# Autodesk Inventor assembly: Intake
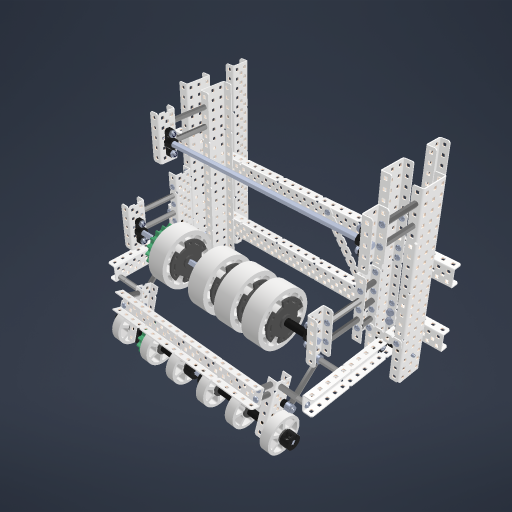
[picture p0: Inventor's stored thumbnail of the model, 512x512]
Saved by Autodesk Inventor 2023 (Build 270158000, 158)
## iProperties
Created: 2022-09-02
Part Number: Intake
Document SubType Name: Assembly
Designer: alex
Author: alex
## Documents named in this file (43)
- C:\Users\alex\Documents\GitHub\4067X_spin_up_cad\Mechanism\Intake.iam
- C:\Users\alex\Documents\GitHub\4067X_spin_up_cad\Library\Structure\Standoff\Standoff 1.00.ipt
- C:\Users\alex\Documents\GitHub\4067X_spin_up_cad\Library\Structure\Standoff.ipt
- C:\Users\alex\Documents\GitHub\4067X_spin_up_cad\Library\Structure\Hardware\Screw Steel - Star\SScrew Star Smooth .290.ipt
- C:\Users\alex\Documents\GitHub\4067X_spin_up_cad\Library\Structure\Hardware\Screw Steel - Star.ipt
- C:\Users\alex\Documents\GitHub\4067X_spin_up_cad\Library\Structure\Standoff\Standoff .50.ipt
- C:\Users\alex\Documents\GitHub\4067X_spin_up_cad\Library\Motion\Spacers\Spacer Nylon .375 OD.ipt
- C:\Users\alex\Documents\GitHub\4067X_spin_up_cad\Library\Structure\Hardware\Nut Keps.ipt
- C:\Users\alex\Documents\GitHub\4067X_spin_up_cad\Library\Structure\Hardware\Screw Steel - Star\SScrew Star Smooth .375.ipt
- C:\Users\alex\Documents\GitHub\4067X_spin_up_cad\Library\Structure\C-Channels\Aluminum 1x3x1\Alu C 1x3x1x20.ipt
- C:\Users\alex\Documents\GitHub\4067X_spin_up_cad\Library\Structure\C-Channels\Aluminum 1x3x1\Alu C 1x3x1x5.ipt
- C:\Users\alex\Documents\GitHub\4067X_spin_up_cad\Library\Structure\C-Channels\Aluminum 1x2x1\Alu C 1x2x1x35.ipt
- C:\Users\alex\Documents\GitHub\4067X_spin_up_cad\Library\Structure\Plates\Aluminum\VEX Plates\Alu Plate VEX 1x11.ipt
- C:\Users\alex\Documents\GitHub\4067X_spin_up_cad\Library\Structure\Standoff\Standoff 2.00.ipt
- C:\Users\alex\Documents\GitHub\4067X_spin_up_cad\Library\Structure\C-Channels\Aluminum 1x2x1\Alu C 1x2x1x5.ipt
- C:\Users\alex\Documents\GitHub\4067X_spin_up_cad\Library\Structure\C-Channels\Aluminum 1x2x1\Alu C 1x2x1x7.ipt
- C:\Users\alex\Documents\GitHub\4067X_spin_up_cad\Library\Structure\Standoff\Standoff .75.ipt
- C:\Users\alex\Documents\GitHub\4067X_spin_up_cad\Library\Motion\Spacers\Spacer Nylon .375 OD\NSpacer .375 OD x .125.ipt
- C:\Users\alex\Documents\GitHub\4067X_spin_up_cad\Library\Motion\Shaft HS\HS Bearing Flat.ipt
- C:\Users\alex\Documents\GitHub\4067X_spin_up_cad\Library\Structure\Hardware\Nut Thin Nylock.ipt
- C:\Users\alex\Documents\GitHub\4067X_spin_up_cad\Library\Structure\Hardware\Screw Steel - Star\SScrew Star Smooth .500.ipt
- C:\Users\alex\Documents\GitHub\4067X_spin_up_cad\Library\Motion\Shaft HS\Shaft HS\Shaft HS 12.0 in.ipt
- C:\Users\alex\Documents\GitHub\4067X_spin_up_cad\Library\Motion\Shaft HS\Shaft HS.ipt
- C:\Users\alex\Documents\GitHub\4067X_spin_up_cad\Library\Motion\Shaft HS\HS Spacer.ipt
- C:\Users\alex\Documents\GitHub\4067X_spin_up_cad\3FlexWheel.iam
- C:\Users\alex\Documents\GitHub\4067X_spin_up_cad\Library\Motion\Shaft HS\HS Spacer\HSpacer .2500.ipt
- C:\Users\alex\Documents\GitHub\4067X_spin_up_cad\Library\Motion\Sprockets\HS 18T Sprocket, No Insert.ipt
- C:\Users\alex\Documents\GitHub\4067X_spin_up_cad\Library\Structure\Hardware\Screw Steel - Star\SScrew Star Smooth 2.250.ipt
- C:\Users\alex\Documents\GitHub\4067X_spin_up_cad\Mechanism\FloatingIntake.iam
- C:\Users\alex\Documents\GitHub\4067X_spin_up_cad\Library\Motion\Spacers\Spacer Nylon .375 OD\NSpacer .375 OD x .375.ipt
- C:\Users\alex\Documents\GitHub\4067X_spin_up_cad\Library\Motion\Spacers\Washer Steel\SWasher .375 OD x .015625.ipt
- C:\Users\alex\Documents\GitHub\4067X_spin_up_cad\Library\Motion\Spacers\Washer Steel.ipt
- C:\Users\alex\Documents\GitHub\4067X_spin_up_cad\Library\Motion\1-Post Bearing Flat Hex Retainer.ipt
- C:\Users\alex\Documents\GitHub\4067X_spin_up_cad\Library\Structure\Hardware\Nut Nylock.ipt
- C:\Users\alex\Documents\GitHub\4067X_spin_up_cad\Library\Motion\Spacers\Spacer Nylon .375 OD\NSpacer .375 OD x .500.ipt
- C:\Users\alex\Documents\GitHub\4067X_spin_up_cad\Library\Motion\Spacers\Washer Teflon\TWasher .375 OD x .06250.ipt
- C:\Users\alex\Documents\GitHub\4067X_spin_up_cad\Library\Motion\Spacers\Washer Teflon.ipt
- C:\Users\alex\Documents\GitHub\4067X_spin_up_cad\Library\Motion\Shaft HS\HS Shaft Collar.ipt
- C:\Users\alex\Documents\GitHub\4067X_spin_up_cad\Library\Motion\Shaft HS\HS Spacer\HSpacer .5000.ipt
- C:\Users\alex\Documents\GitHub\4067X_spin_up_cad\Library\Motion\Shaft HS\HS Spacer\HSpacer .1250.ipt
- C:\Users\alex\Documents\GitHub\4067X_spin_up_cad\Library\Structure\C-Channels\Aluminum 1x2x1\Alu C 1x2x1x21.ipt
- C:\Users\alex\Documents\GitHub\4067X_spin_up_cad\Library\Structure\Hardware\Screw Steel - Star\SScrew Star Smooth .750.ipt
- C:\Users\alex\Documents\GitHub\4067X_spin_up_cad\Library\Structure\Plates\Aluminum\VEX Plates\Alu Plate VEX 1x4.ipt
## Components (166 placed, 35 different names)
1. Alu C 1x2x1x35:1 — Insert:150, Insert:151, Insert:218, Insert:219, Insert:236, Insert:237, Insert:400, Insert:401, Insert:419, Insert:420, Insert:448, Insert:449, Insert:458, Insert:459, Insert:469, Insert:475, Insert:504, Insert:505
2. Standoff 1.00:16 — Insert:110, Insert:404
3. Standoff .50:17 — Insert:110, Insert:496
4. Standoff 1.00:18 — Insert:405
5. Standoff .50:19 — Insert:497
6. Standoff 1.00:20 — Insert:454
7. Standoff .50:21 — Insert:500
8. Standoff 1.00:22 — Insert:455
9. Standoff .50:23 — Insert:501
10. Alu C 1x3x1x5:2 — Insert:150, Insert:151, Insert:217, Insert:220, Insert:221, Insert:428, Mate:67, Insert:429, Insert:439
11. Nut Keps:12 — Insert:217
12. SScrew Star Smooth .290:52 — Insert:218
13. SScrew Star Smooth .290:53 — Insert:219
14. Nut Keps:13 — Insert:220
15. Nut Keps:14 — Insert:221
16. SScrew Star Smooth .290:62 — Insert:236
17. SScrew Star Smooth .290:63 — Insert:237
18. Alu C 1x2x1x35:2 — Insert:417, Insert:418, Insert:467, Insert:470, Insert:476, Insert:481, Insert:482, Insert:535, Insert:536
19. SScrew Star Smooth .290:86 — Insert:456
20. SScrew Star Smooth .290:90 — Insert:407
21. SScrew Star Smooth .290:91 — Insert:406
22. Alu C 1x2x1x5:2 — Insert:334, Insert:335, Insert:338, Insert:339, Insert:488, Mate:72, Insert:489, Insert:490
23. Standoff 2.00:27 — Insert:334, Insert:382
24. Standoff 2.00:28 — Insert:335, Insert:381
25. SScrew Star Smooth .290:102 — Insert:338
26. SScrew Star Smooth .290:103 — Insert:339
27. Alu C 1x2x1x7:1 — Insert:345, Insert:346, Insert:347, Insert:348, Insert:349, Insert:358, Insert:359, Insert:360, Insert:361, Insert:362, Insert:381, Insert:382, Insert:522
28. SScrew Star Smooth .290:106 — Insert:345
29. SScrew Star Smooth .290:107 — Insert:346
30. Standoff .75:29 — Insert:347, Insert:355
31. Standoff .75:30 — Insert:348, Insert:356
32. Standoff .75:31 — Insert:349, Insert:357
33. NSpacer .375 OD x .125:13 — Insert:355
34. NSpacer .375 OD x .125:14 — Insert:356
35. NSpacer .375 OD x .125:15 — Insert:357
36. SScrew Star Smooth .375:111 — Insert:358
37. SScrew Star Smooth .375:112 — Insert:359
38. SScrew Star Smooth .375:113 — Insert:360
39. SScrew Star Smooth .290:114 — Insert:361
40. SScrew Star Smooth .290:115 — Insert:362
41. Alu C 1x2x1x5:3 — Insert:485, Mate:71, Insert:486, Insert:487, Flush:1
42. Standoff 2.00:32 — Insert:384
43. Standoff 2.00:33 — Insert:383
44. SScrew Star Smooth .290:116
45. SScrew Star Smooth .290:117
46. Alu C 1x2x1x7:2 — Insert:383, Insert:384, Insert:521, Mate:77, Insert:528, Insert:529
47. SScrew Star Smooth .290:118
48. Standoff .75:34
49. Standoff .75:35
50. Standoff .75:36
51. NSpacer .375 OD x .125:16
52. NSpacer .375 OD x .125:17
53. NSpacer .375 OD x .125:18
54. SScrew Star Smooth .375:120
55. SScrew Star Smooth .375:121
56. SScrew Star Smooth .375:122
57. SScrew Star Smooth .290:123
58. SScrew Star Smooth .290:124
59. Shaft HS 12.0 in:1 — Mate:43, Angle:1, Angle:2, Mate:47, Mate:50, Mate:51, Mate:53, Angle:3, Mate:57, Angle:4, Mate:58, Angle:5, Mate:73, Flush:1, Mate:74
60. 3FlexWheel:1 [sub-assembly] — Mate:43, Angle:1, Mate:48, Mate:76
61. 3FlexWheel:2 [sub-assembly] — Angle:2, Mate:49, Mate:50, Mate:52
62. HSpacer .2500:2 — Mate:47, Mate:48, Mate:49
63. HSpacer .2500:3 — Mate:51, Mate:52, Mate:54
64. 3FlexWheel:3 [sub-assembly] — Mate:53, Angle:3, Mate:54
65. 3FlexWheel:4 [sub-assembly] — Mate:58, Angle:5, Mate:59
66. HS 18T Sprocket, No Insert:1 — Mate:57, Angle:4, Mate:59, Flush:2, Mate:75
67. Alu C 1x3x1x20:3 — Insert:400, Insert:401, Insert:404, Insert:405, Insert:406, Insert:407, Insert:413, Insert:414, Insert:416, Insert:460, Insert:461, Insert:467, Insert:468, Insert:521, Insert:527, Insert:530, Insert:531, Insert:532
68. SScrew Star Smooth 2.250:132 — Insert:413
69. Nut Keps:43 — Insert:414, Insert:433
70. SScrew Star Smooth .290:134 — Insert:416
71. Nut Keps:44 — Insert:417
72. Nut Keps:45 — Insert:418
73. Alu C 1x3x1x20:4 — Insert:419, Insert:420, Insert:421, Insert:424, Mate:66, Insert:446, Insert:452, Insert:453, Insert:454, Insert:455, Insert:456, Insert:457, Insert:462, Insert:463, Insert:479, Insert:480, Insert:522, Insert:523
74. SScrew Star Smooth 2.250:135 — Insert:421, Mate:65
75. Nut Keps:46 — Insert:424, Insert:425
76. FloatingIntake:1 [sub-assembly] — Mate:65, Mate:66, Insert:430, Insert:435, Flush:2
77. NSpacer .375 OD x .375:19 — Insert:425, Insert:426
78. SWasher .375 OD x .015625:1 — Insert:426
79. 1-Post Bearing Flat Hex Retainer:1 — Insert:428, Mate:67
80. Nut Nylock:1
81. SScrew Star Smooth .375:136 — Insert:429
82. NSpacer .375 OD x .500:20 — Insert:430, Insert:431
83. NSpacer .375 OD x .375:21 — Insert:431
84. NSpacer .375 OD x .375:22 — Insert:433
85. SWasher .375 OD x .015625:2
86. NSpacer .375 OD x .500:23 — Insert:435
87. NSpacer .375 OD x .375:24
88. TWasher .375 OD x .06250:1 — Insert:439
89. SScrew Star Smooth .375:138
90. TWasher .375 OD x .06250:2 — Insert:524, Insert:525
91. SScrew Star Smooth .375:139
92. Nut Keps:47 — Insert:446
93. SScrew Star Smooth .290:141 — Insert:448
94. SScrew Star Smooth .290:142 — Insert:449
95. Nut Keps:50 — Insert:452
96. Nut Keps:51 — Insert:453
97. SScrew Star Smooth .290:143 — Insert:457
98. SScrew Star Smooth .290:144 — Insert:458
99. SScrew Star Smooth .290:145 — Insert:459
100. Nut Keps:52 — Insert:460
101. Nut Keps:53 — Insert:461
102. SScrew Star Smooth .290:146 — Insert:462
103. SScrew Star Smooth .290:147 — Insert:463
104. SScrew Star Smooth .290:149 — Insert:468
105. Alu Plate VEX 1x11:4 — Insert:469, Insert:470, Insert:473, Insert:474
106. SScrew Star Smooth .290:152 — Insert:473
107. SScrew Star Smooth .290:153 — Insert:474
108. Nut Keps:54 — Insert:475
109. Nut Keps:55 — Insert:476
110. SScrew Star Smooth .290:154 — Insert:479
111. SScrew Star Smooth .290:155 — Insert:480
112. Nut Keps:58 — Insert:481
113. Nut Keps:59 — Insert:482
114. HS Bearing Flat:3 — Insert:485, Mate:71, Insert:493
115. Nut Thin Nylock:5
116. Nut Thin Nylock:6
117. SScrew Star Smooth .500:156 — Insert:486
118. SScrew Star Smooth .500:157 — Insert:487
119. HS Bearing Flat:4 — Insert:488, Mate:72, Mate:73, Insert:491, Insert:492
120. SScrew Star Smooth .500:158 — Insert:489
121. SScrew Star Smooth .500:159 — Insert:490
122. Nut Thin Nylock:7 — Insert:491
123. Nut Thin Nylock:8 — Insert:492
124. HS Shaft Collar:1 — Mate:74, Mate:75
125. HSpacer .5000:4 — Insert:493, Insert:494
126. HSpacer .5000:5 — Insert:494, Insert:495
127. HSpacer .1250:6 — Insert:495, Mate:76
128. Alu C 1x2x1x21:1 — Insert:496, Insert:497, Insert:498, Insert:499
129. SScrew Star Smooth .750:160 — Insert:498
130. SScrew Star Smooth .750:161 — Insert:499
131. Alu C 1x2x1x21:2 — Insert:500, Insert:501, Insert:502, Insert:503
132. SScrew Star Smooth .750:162 — Insert:502
133. SScrew Star Smooth .750:163 — Insert:503
134. Alu C 1x3x1x20:5 — Insert:504, Insert:505, Insert:506, Insert:507, Insert:508, Insert:525, Insert:541, Insert:542
135. Nut Keps:60 — Insert:506
136. Nut Keps:61 — Insert:507
137. Nut Keps:62 — Insert:508
138. Alu C 1x2x1x5:5 — Insert:545, Mate:78, Insert:546, Insert:547
139. Standoff 2.00:39 — Insert:541
140. Standoff 2.00:40 — Insert:542
141. SScrew Star Smooth .290:166
142. SScrew Star Smooth .290:167
143. SScrew Star Smooth .290:168 — Insert:523
144. Alu Plate VEX 1x4:1 — Insert:524, Mate:77, Insert:526
145. SScrew Star Smooth .375:169 — Insert:526
146. Nut Keps:64 — Insert:527
147. SScrew Star Smooth .290:170 — Insert:528
148. SScrew Star Smooth .290:171 — Insert:529
149. Nut Keps:65 — Insert:530
150. Nut Keps:66 — Insert:531
151. Nut Keps:67 — Insert:532
152. Alu C 1x3x1x20:6 — Insert:535, Insert:536, Insert:539, Insert:540
153. Alu C 1x2x1x5:6 — Insert:550, Mate:79, Insert:551, Insert:552, Flush:3
154. Standoff 2.00:41 — Insert:539
155. Standoff 2.00:42 — Insert:540
156. HS Bearing Flat:5 — Insert:545, Mate:78
157. Nut Thin Nylock:9
158. Nut Thin Nylock:10
159. SScrew Star Smooth .500:172 — Insert:546
160. SScrew Star Smooth .500:173 — Insert:547
161. HS Bearing Flat:6 — Insert:550, Mate:79, Mate:80
162. Nut Thin Nylock:11
163. Nut Thin Nylock:12
164. SScrew Star Smooth .500:174 — Insert:551
165. SScrew Star Smooth .500:175 — Insert:552
166. Shaft HS 12.0 in:2 — Mate:80, Flush:3
## Relationships (197: Insert 164, Mate 25, Angle 5, Flush 3)
- Insert:110: Standoff 1.00:16 ↔ Standoff .50:17
- [Insert]: Standoff 1.00:18 ↔ Standoff .50:19
- [Insert]: Standoff 1.00:20 ↔ Standoff .50:21
- [Insert]: Standoff 1.00:22 ↔ Standoff .50:23
- Insert:150: Alu C 1x2x1x35:1 ↔ Alu C 1x3x1x5:2
- Insert:151: Alu C 1x2x1x35:1 ↔ Alu C 1x3x1x5:2
- Insert:217: Alu C 1x3x1x5:2 ↔ Nut Keps:12
- Insert:218: Alu C 1x2x1x35:1 ↔ SScrew Star Smooth .290:52
- Insert:219: Alu C 1x2x1x35:1 ↔ SScrew Star Smooth .290:53
- Insert:220: Alu C 1x3x1x5:2 ↔ Nut Keps:13
- Insert:221: Alu C 1x3x1x5:2 ↔ Nut Keps:14
- Insert:236: Alu C 1x2x1x35:1 ↔ SScrew Star Smooth .290:62
- Insert:237: Alu C 1x2x1x35:1 ↔ SScrew Star Smooth .290:63
- Insert:334: Alu C 1x2x1x5:2 ↔ Standoff 2.00:27
- Insert:335: Alu C 1x2x1x5:2 ↔ Standoff 2.00:28
- Insert:338: Alu C 1x2x1x5:2 ↔ SScrew Star Smooth .290:102
- Insert:339: Alu C 1x2x1x5:2 ↔ SScrew Star Smooth .290:103
- Insert:345: Alu C 1x2x1x7:1 ↔ SScrew Star Smooth .290:106
- Insert:346: Alu C 1x2x1x7:1 ↔ SScrew Star Smooth .290:107
- Insert:347: Alu C 1x2x1x7:1 ↔ Standoff .75:29
- Insert:348: Alu C 1x2x1x7:1 ↔ Standoff .75:30
- Insert:349: Alu C 1x2x1x7:1 ↔ Standoff .75:31
- Insert:355: Standoff .75:29 ↔ NSpacer .375 OD x .125:13
- Insert:356: Standoff .75:30 ↔ NSpacer .375 OD x .125:14
- Insert:357: Standoff .75:31 ↔ NSpacer .375 OD x .125:15
- Insert:358: Alu C 1x2x1x7:1 ↔ SScrew Star Smooth .375:111
- Insert:359: Alu C 1x2x1x7:1 ↔ SScrew Star Smooth .375:112
- Insert:360: Alu C 1x2x1x7:1 ↔ SScrew Star Smooth .375:113
- Insert:361: Alu C 1x2x1x7:1 ↔ SScrew Star Smooth .290:114
- Insert:362: Alu C 1x2x1x7:1 ↔ SScrew Star Smooth .290:115
- [Insert]: Alu C 1x2x1x5:3 ↔ Standoff 2.00:32
- [Insert]: Alu C 1x2x1x5:3 ↔ Standoff 2.00:33
- [Insert]: Alu C 1x2x1x5:3 ↔ SScrew Star Smooth .290:116
- [Insert]: Alu C 1x2x1x5:3 ↔ SScrew Star Smooth .290:117
- [Insert]: Alu C 1x2x1x7:2 ↔ SScrew Star Smooth .290:118
- [Insert]: Alu C 1x2x1x7:2 ↔ Standoff .75:34
- [Insert]: Alu C 1x2x1x7:2 ↔ Standoff .75:35
- [Insert]: Alu C 1x2x1x7:2 ↔ Standoff .75:36
- [Insert]: Standoff .75:34 ↔ NSpacer .375 OD x .125:16
- [Insert]: Standoff .75:35 ↔ NSpacer .375 OD x .125:17
- [Insert]: Standoff .75:36 ↔ NSpacer .375 OD x .125:18
- [Insert]: Alu C 1x2x1x7:2 ↔ SScrew Star Smooth .375:120
- [Insert]: Alu C 1x2x1x7:2 ↔ SScrew Star Smooth .375:121
- [Insert]: Alu C 1x2x1x7:2 ↔ SScrew Star Smooth .375:122
- [Insert]: Alu C 1x2x1x7:2 ↔ SScrew Star Smooth .290:123
- [Insert]: Alu C 1x2x1x7:2 ↔ SScrew Star Smooth .290:124
- Insert:381: Standoff 2.00:28 ↔ Alu C 1x2x1x7:1
- Insert:382: Standoff 2.00:27 ↔ Alu C 1x2x1x7:1
- Insert:383: Standoff 2.00:33 ↔ Alu C 1x2x1x7:2
- Insert:384: Standoff 2.00:32 ↔ Alu C 1x2x1x7:2
- Mate:43: Shaft HS 12.0 in:1 ↔ 3FlexWheel:1
- Angle:1 (0 deg): Shaft HS 12.0 in:1 ↔ 3FlexWheel:1
- Angle:2 (0 deg): Shaft HS 12.0 in:1 ↔ 3FlexWheel:2
- Mate:47: Shaft HS 12.0 in:1 ↔ HSpacer .2500:2
- Mate:48: 3FlexWheel:1 ↔ HSpacer .2500:2
- Mate:49: 3FlexWheel:2 ↔ HSpacer .2500:2
- Mate:50: Shaft HS 12.0 in:1 ↔ 3FlexWheel:2
- Mate:51: Shaft HS 12.0 in:1 ↔ HSpacer .2500:3
- Mate:52: 3FlexWheel:2 ↔ HSpacer .2500:3
- Mate:53: Shaft HS 12.0 in:1 ↔ 3FlexWheel:3
- Angle:3 (0 deg): Shaft HS 12.0 in:1 ↔ 3FlexWheel:3
- Mate:54: HSpacer .2500:3 ↔ 3FlexWheel:3
- Mate:57: Shaft HS 12.0 in:1 ↔ HS 18T Sprocket, No Insert:1
- Angle:4 (0 deg): Shaft HS 12.0 in:1 ↔ HS 18T Sprocket, No Insert:1
- Mate:58: Shaft HS 12.0 in:1 ↔ 3FlexWheel:4
- Angle:5 (0 deg): Shaft HS 12.0 in:1 ↔ 3FlexWheel:4
- Mate:59: 3FlexWheel:4 ↔ HS 18T Sprocket, No Insert:1
- Insert:400: Alu C 1x2x1x35:1 ↔ Alu C 1x3x1x20:3
- Insert:401: Alu C 1x2x1x35:1 ↔ Alu C 1x3x1x20:3
- Insert:404: Standoff 1.00:16 ↔ Alu C 1x3x1x20:3
- Insert:405: Standoff 1.00:18 ↔ Alu C 1x3x1x20:3
- Insert:406: SScrew Star Smooth .290:91 ↔ Alu C 1x3x1x20:3
- Insert:407: SScrew Star Smooth .290:90 ↔ Alu C 1x3x1x20:3
- Insert:413: Alu C 1x3x1x20:3 ↔ SScrew Star Smooth 2.250:132
- Insert:414: Alu C 1x3x1x20:3 ↔ Nut Keps:43
- Insert:416: Alu C 1x3x1x20:3 ↔ SScrew Star Smooth .290:134
- Insert:417: Alu C 1x2x1x35:2 ↔ Nut Keps:44
- Insert:418: Alu C 1x2x1x35:2 ↔ Nut Keps:45
- Insert:419: Alu C 1x2x1x35:1 ↔ Alu C 1x3x1x20:4
- Insert:420: Alu C 1x2x1x35:1 ↔ Alu C 1x3x1x20:4
- Insert:421: Alu C 1x3x1x20:4 ↔ SScrew Star Smooth 2.250:135
- Insert:424: Alu C 1x3x1x20:4 ↔ Nut Keps:46
- Mate:65: SScrew Star Smooth 2.250:135 ↔ FloatingIntake:1
- Mate:66 (13.6398 mm): Alu C 1x3x1x20:4 ↔ FloatingIntake:1
- Insert:425: Nut Keps:46 ↔ NSpacer .375 OD x .375:19
- Insert:426: NSpacer .375 OD x .375:19 ↔ SWasher .375 OD x .015625:1
- [Insert]: 1-Post Bearing Flat Hex Retainer:1 ↔ Nut Nylock:1
- Insert:428: Alu C 1x3x1x5:2 ↔ 1-Post Bearing Flat Hex Retainer:1
- Mate:67: Alu C 1x3x1x5:2 ↔ 1-Post Bearing Flat Hex Retainer:1
- Insert:429: Alu C 1x3x1x5:2 ↔ SScrew Star Smooth .375:136
- Insert:430: FloatingIntake:1 ↔ NSpacer .375 OD x .500:20
- Insert:431: NSpacer .375 OD x .500:20 ↔ NSpacer .375 OD x .375:21
- [Insert]: NSpacer .375 OD x .375:22 ↔ SWasher .375 OD x .015625:2
- Insert:433: Nut Keps:43 ↔ NSpacer .375 OD x .375:22
- [Insert]: NSpacer .375 OD x .500:23 ↔ NSpacer .375 OD x .375:24
- Insert:435: FloatingIntake:1 ↔ NSpacer .375 OD x .500:23
- Insert:439: Alu C 1x3x1x5:2 ↔ TWasher .375 OD x .06250:1
- Insert:446: Alu C 1x3x1x20:4 ↔ Nut Keps:47
- Insert:448: Alu C 1x2x1x35:1 ↔ SScrew Star Smooth .290:141
- Insert:449: Alu C 1x2x1x35:1 ↔ SScrew Star Smooth .290:142
- Insert:452: Alu C 1x3x1x20:4 ↔ Nut Keps:50
- Insert:453: Alu C 1x3x1x20:4 ↔ Nut Keps:51
- Insert:454: Standoff 1.00:20 ↔ Alu C 1x3x1x20:4
- Insert:455: Standoff 1.00:22 ↔ Alu C 1x3x1x20:4
- Insert:456: SScrew Star Smooth .290:86 ↔ Alu C 1x3x1x20:4
- Insert:457: Alu C 1x3x1x20:4 ↔ SScrew Star Smooth .290:143
- Insert:458: Alu C 1x2x1x35:1 ↔ SScrew Star Smooth .290:144
- Insert:459: Alu C 1x2x1x35:1 ↔ SScrew Star Smooth .290:145
- Insert:460: Alu C 1x3x1x20:3 ↔ Nut Keps:52
- Insert:461: Alu C 1x3x1x20:3 ↔ Nut Keps:53
- Insert:462: Alu C 1x3x1x20:4 ↔ SScrew Star Smooth .290:146
- Insert:463: Alu C 1x3x1x20:4 ↔ SScrew Star Smooth .290:147
- Insert:467: Alu C 1x2x1x35:2 ↔ Alu C 1x3x1x20:3
- Insert:468: Alu C 1x3x1x20:3 ↔ SScrew Star Smooth .290:149
- Insert:469: Alu C 1x2x1x35:1 ↔ Alu Plate VEX 1x11:4
- Insert:470: Alu C 1x2x1x35:2 ↔ Alu Plate VEX 1x11:4
- Insert:473: Alu Plate VEX 1x11:4 ↔ SScrew Star Smooth .290:152
- Insert:474: Alu Plate VEX 1x11:4 ↔ SScrew Star Smooth .290:153
- Insert:475: Alu C 1x2x1x35:1 ↔ Nut Keps:54
- Insert:476: Alu C 1x2x1x35:2 ↔ Nut Keps:55
- Insert:479: Alu C 1x3x1x20:4 ↔ SScrew Star Smooth .290:154
- Insert:480: Alu C 1x3x1x20:4 ↔ SScrew Star Smooth .290:155
- Insert:481: Alu C 1x2x1x35:2 ↔ Nut Keps:58
- Insert:482: Alu C 1x2x1x35:2 ↔ Nut Keps:59
- [Insert]: HS Bearing Flat:3 ↔ Nut Thin Nylock:5
- [Insert]: HS Bearing Flat:3 ↔ Nut Thin Nylock:6
- Insert:485: Alu C 1x2x1x5:3 ↔ HS Bearing Flat:3
- Mate:71: Alu C 1x2x1x5:3 ↔ HS Bearing Flat:3
- Insert:486: Alu C 1x2x1x5:3 ↔ SScrew Star Smooth .500:156
- Insert:487: Alu C 1x2x1x5:3 ↔ SScrew Star Smooth .500:157
- Insert:488: Alu C 1x2x1x5:2 ↔ HS Bearing Flat:4
- Mate:72: Alu C 1x2x1x5:2 ↔ HS Bearing Flat:4
- Insert:489: Alu C 1x2x1x5:2 ↔ SScrew Star Smooth .500:158
- Insert:490: Alu C 1x2x1x5:2 ↔ SScrew Star Smooth .500:159
- Mate:73: Shaft HS 12.0 in:1 ↔ HS Bearing Flat:4
- Insert:491: HS Bearing Flat:4 ↔ Nut Thin Nylock:7
- Insert:492: HS Bearing Flat:4 ↔ Nut Thin Nylock:8
- Flush:1 (-6.0198 mm): Alu C 1x2x1x5:3 ↔ Shaft HS 12.0 in:1
- Flush:2: HS 18T Sprocket, No Insert:1 ↔ FloatingIntake:1
- Mate:74: Shaft HS 12.0 in:1 ↔ HS Shaft Collar:1
- Mate:75: HS 18T Sprocket, No Insert:1 ↔ HS Shaft Collar:1
- Insert:493: HS Bearing Flat:3 ↔ HSpacer .5000:4
- Insert:494: HSpacer .5000:4 ↔ HSpacer .5000:5
- Insert:495: HSpacer .5000:5 ↔ HSpacer .1250:6
- Mate:76: 3FlexWheel:1 ↔ HSpacer .1250:6
- Insert:496: Standoff .50:17 ↔ Alu C 1x2x1x21:1
- Insert:497: Standoff .50:19 ↔ Alu C 1x2x1x21:1
- Insert:498: Alu C 1x2x1x21:1 ↔ SScrew Star Smooth .750:160
- Insert:499: Alu C 1x2x1x21:1 ↔ SScrew Star Smooth .750:161
- Insert:500: Standoff .50:21 ↔ Alu C 1x2x1x21:2
- Insert:501: Standoff .50:23 ↔ Alu C 1x2x1x21:2
- Insert:502: Alu C 1x2x1x21:2 ↔ SScrew Star Smooth .750:162
- Insert:503: Alu C 1x2x1x21:2 ↔ SScrew Star Smooth .750:163
- Insert:504: Alu C 1x2x1x35:1 ↔ Alu C 1x3x1x20:5
- Insert:505: Alu C 1x2x1x35:1 ↔ Alu C 1x3x1x20:5
- Insert:506: Alu C 1x3x1x20:5 ↔ Nut Keps:60
- Insert:507: Alu C 1x3x1x20:5 ↔ Nut Keps:61
- Insert:508: Alu C 1x3x1x20:5 ↔ Nut Keps:62
- [Insert]: Alu C 1x2x1x5:5 ↔ Standoff 2.00:39
- [Insert]: Alu C 1x2x1x5:5 ↔ Standoff 2.00:40
- [Insert]: Alu C 1x2x1x5:5 ↔ SScrew Star Smooth .290:166
- [Insert]: Alu C 1x2x1x5:5 ↔ SScrew Star Smooth .290:167
- Insert:521: Alu C 1x2x1x7:2 ↔ Alu C 1x3x1x20:3
- Insert:522: Alu C 1x2x1x7:1 ↔ Alu C 1x3x1x20:4
- Insert:523: Alu C 1x3x1x20:4 ↔ SScrew Star Smooth .290:168
- Insert:524: TWasher .375 OD x .06250:2 ↔ Alu Plate VEX 1x4:1
- Insert:525: TWasher .375 OD x .06250:2 ↔ Alu C 1x3x1x20:5
- Mate:77: Alu C 1x2x1x7:2 ↔ Alu Plate VEX 1x4:1
- Insert:526: Alu Plate VEX 1x4:1 ↔ SScrew Star Smooth .375:169
- Insert:527: Alu C 1x3x1x20:3 ↔ Nut Keps:64
- Insert:528: Alu C 1x2x1x7:2 ↔ SScrew Star Smooth .290:170
- Insert:529: Alu C 1x2x1x7:2 ↔ SScrew Star Smooth .290:171
- Insert:530: Alu C 1x3x1x20:3 ↔ Nut Keps:65
- Insert:531: Alu C 1x3x1x20:3 ↔ Nut Keps:66
- Insert:532: Alu C 1x3x1x20:3 ↔ Nut Keps:67
- Insert:535: Alu C 1x2x1x35:2 ↔ Alu C 1x3x1x20:6
- Insert:536: Alu C 1x2x1x35:2 ↔ Alu C 1x3x1x20:6
- [Insert]: Alu C 1x2x1x5:6 ↔ Standoff 2.00:41
- [Insert]: Alu C 1x2x1x5:6 ↔ Standoff 2.00:42
- Insert:539: Alu C 1x3x1x20:6 ↔ Standoff 2.00:41
- Insert:540: Alu C 1x3x1x20:6 ↔ Standoff 2.00:42
- Insert:541: Alu C 1x3x1x20:5 ↔ Standoff 2.00:39
- Insert:542: Alu C 1x3x1x20:5 ↔ Standoff 2.00:40
- [Insert]: HS Bearing Flat:5 ↔ Nut Thin Nylock:9
- [Insert]: HS Bearing Flat:5 ↔ Nut Thin Nylock:10
- Insert:545: Alu C 1x2x1x5:5 ↔ HS Bearing Flat:5
- Mate:78: Alu C 1x2x1x5:5 ↔ HS Bearing Flat:5
- Insert:546: Alu C 1x2x1x5:5 ↔ SScrew Star Smooth .500:172
- Insert:547: Alu C 1x2x1x5:5 ↔ SScrew Star Smooth .500:173
- [Insert]: HS Bearing Flat:6 ↔ Nut Thin Nylock:11
- [Insert]: HS Bearing Flat:6 ↔ Nut Thin Nylock:12
- Insert:550: Alu C 1x2x1x5:6 ↔ HS Bearing Flat:6
- Mate:79: Alu C 1x2x1x5:6 ↔ HS Bearing Flat:6
- Insert:551: Alu C 1x2x1x5:6 ↔ SScrew Star Smooth .500:174
- Insert:552: Alu C 1x2x1x5:6 ↔ SScrew Star Smooth .500:175
- Mate:80: HS Bearing Flat:6 ↔ Shaft HS 12.0 in:2
- Flush:3 (-6.0198 mm): Alu C 1x2x1x5:6 ↔ Shaft HS 12.0 in:2
## Named parameters: d171_d169 = 0 mm, d195_d169 = 0 mm, d197_d195_d169 = 0 mm, d492_d477 = 0 mm, d493_d478 = 0 mm, d494_d484 = 0 mm, d495_d485 = 0 mm, d496_d486 = 0 mm, d497_d487 = 0 mm, d498_d488 = 0 mm, d499_d489 = 0 mm, d500_d490 = 0 mm, d501_d491 = 0 mm, d502_d463 = 0 mm, d503_d464 = 0 mm, d504_d467 = 0 mm, d505_d468 = 0 mm, d506_d474 = 0 mm, d508_d476 = 0 mm, d208_d147 = 0 mm, d606_d599 = 0 mm, d608_d605 = 0 mm, d660_d521_d253_d244 = 0 mm, d661_d522_d520 = 0 mm, d705_d699_d502_d463 = 0 mm, d706_d700_d503_d464 = 0 mm, d707_d701_d504_d467 = 0 mm, d708_d702_d505_d468 = 0 mm, d730_d705_d699_d502_d463 = 0 mm, d731_d706_d700_d503_d464 = 0 mm, d736_d660_d521_d253_d244 = 0 mm, d737_d661_d522_d520 = 0 mm, d742_d736_d660_d521_d253_d244 = 0 mm, d743_d737_d661_d522_d520 = 0 mm
